# Autodesk Inventor assembly: Assembly1
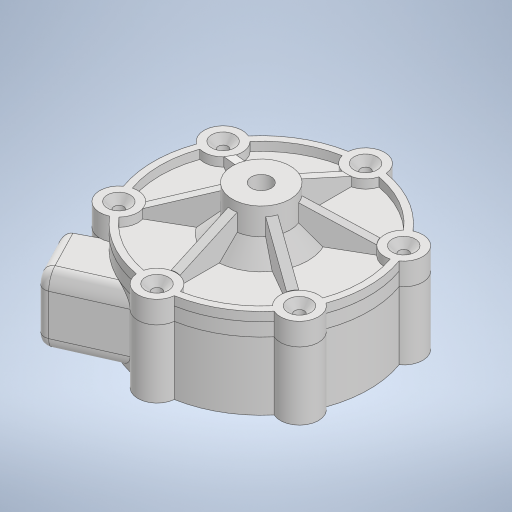
[picture p0: Inventor's stored thumbnail of the model, 512x512]
Saved by Autodesk Inventor 2023.1 (Build 271208000, 208)
## iProperties
Created: 2024-02-14
Part Number: Assembly1
Document SubType Name: Assembly
Designer: USER
Author: USER
## Documents named in this file (5)
- C:\Users\Robot\Documents\WaterPump\Assembly1.iam
- C:\Users\Robot\Documents\WaterPump\Propeller.ipt
- C:\Users\Robot\Documents\WaterPump\Motor.ipt
- C:\Users\Robot\Documents\WaterPump\case.ipt
- C:\Users\Robot\Documents\Vesters3DPrinter\top_cover.ipt
## Components (4 placed, 4 different names)
1. Propeller:1
2. Motor:1 — Flush:1
3. case:1 — Flush:1, Flush:2
4. top_cover:1 — Flush:2, Flush:3
## Relationships (3: Flush 3)
- Flush:1: Motor:1 ↔ case:1
- Flush:2: case:1 ↔ top_cover:1
- Flush:3: top_cover:1
